# Autodesk Inventor assembly: CL4-300
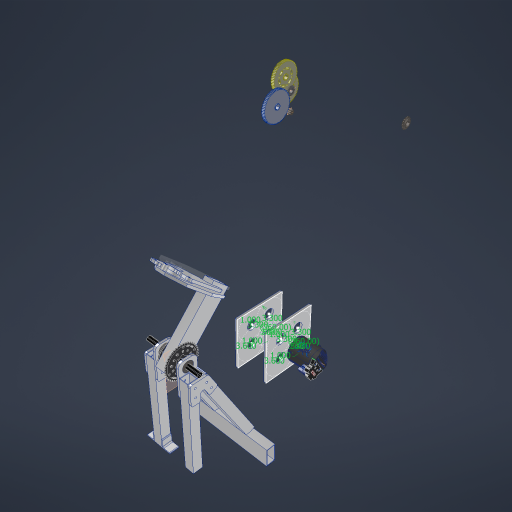
[picture p0: Inventor's stored thumbnail of the model, 512x512]
Saved by Autodesk Inventor 2023.4 (Build 274418000, 418)
## iProperties
Created: 2025-02-04
Part Number: CL4-300
Document SubType Name: Assembly
Designer: brand
Mass: 2767.61 g
Surface Area: 6209.23 cm^2
Volume: 1040.03 cm^3
Density: 2.66107 g/cm^3
Author: brand
## Documents named in this file (15)
- C:\Users\brand\OneDrive\Documents\GitHub\robotics 23\2025-ReefScape---CAD\Climber\CL4\CL4-300.iam
- C:\Users\brand\OneDrive\Documents\GitHub\robotics 23\2025-ReefScape---CAD\Climber\CL4\CL4-200.iam
- C:\Users\brand\OneDrive\Documents\GitHub\robotics 23\2025-ReefScape---CAD\Climber\CL4\CL4-100.iam
- C:\Users\brand\OneDrive\Documents\GitHub\robotics 23\2025-ReefScape---CAD\COMMON PARTS\BEARINGS\0_500_Hex_ID_x_1_125_OD_x_0_313_WD_Flanged_Bearing_v2_217-3875.ipt
- C:\Users\brand\OneDrive\Documents\GitHub\robotics 23\2025-ReefScape---CAD\Climber\CL4\CL4-011.ipt
- C:\Users\brand\OneDrive\Documents\GitHub\robotics 23\2025-ReefScape---CAD\Climber\CL4\CL4-012.ipt
- C:\Users\brand\OneDrive\Documents\GitHub\robotics 23\2025-ReefScape---CAD\Climber\CL4\CL4-013.ipt
- C:\Users\brand\OneDrive\Documents\GitHub\robotics 23\2025-ReefScape---CAD\COMMON PARTS\GEARS\WCP-1006\WCP-1006.ipt
- C:\Users\brand\OneDrive\Documents\GitHub\robotics 23\2025-ReefScape---CAD\COMMON PARTS\GEARS\20dp .5 hex\72t_Aluminum_Spur_Gear_20_DP_1_2_Hex_Bore_217-3576.ipt
- C:\Users\brand\OneDrive\Documents\GitHub\robotics 23\2025-ReefScape---CAD\COMMON PARTS\GEARS\20dp .5 hex\66t_Aluminum_Spur_Gear_20_DP_1_2_Hex_Bore_VersaKeys_217-3223.ipt
- C:\Users\brand\OneDrive\Documents\GitHub\robotics 23\2025-ReefScape---CAD\COMMON PARTS\GEARS\20dp .5 hex\20t_Aluminum_Spur_Gear_20_DP_1_2_Hex_Bore_217-2702.ipt
- C:\Users\brand\OneDrive\Documents\GitHub\robotics 23\2025-ReefScape---CAD\COMMON PARTS\SPROCKETS\25\WCP-0967 42t 25_chain.ipt
- C:\Users\brand\OneDrive\Documents\GitHub\robotics 23\2025-ReefScape---CAD\COMMON PARTS\SPROCKETS\25\14t Steel Double Hub Sprocket (#25 Chain, 12 Hex Bore)\14t Steel Double Hub Sprocket (#25 Chain, 12 Hex Bore).ipt
- C:\Users\brand\OneDrive\Documents\GitHub\robotics 23\2025-ReefScape---CAD\COMMON PARTS\MOTORS\Kracken with Cover and Boards.iam
- C:\Users\brand\OneDrive\Documents\GitHub\robotics 23\2025-ReefScape---CAD\Climber\CL4\CL4-014.ipt
## Components (19 placed, 14 different names)
1. CL4-200:1 [sub-assembly] — Insert:1, Insert:2, Angle:1, Flush:1, Mate:3, Mate:6, Mate:4, Mate:5, Flush:7, Flush:8, Flush:9, Flush:10, Mate:8
2. CL4-100:1 [sub-assembly] — Mate:2, Angle:1, Flush:1, Mate:13, Mate:14
3. 0_500_Hex_ID_x_1_125_OD_x_0_313_WD_Flanged_Bearing_v2_217-3875:1 — Insert:1, Mate:1
4. 0_500_Hex_ID_x_1_125_OD_x_0_313_WD_Flanged_Bearing_v2_217-3875:2 — Insert:2
5. CL4-011:1 — Mate:1, Mate:2
6. CL4-012:1 — Mate:3, Mate:6, Mate:7, Flush:11
7. CL4-013:1 — Mate:4, Flush:7, Flush:8
8. CL4-013:2 — Mate:5, Flush:9, Flush:10
9. CL4-013:3 — Mate:7, Flush:11, Mate:8
10. WCP-1006:1
11. 72t_Aluminum_Spur_Gear_20_DP_1_2_Hex_Bore_217-3576:1
12. 66t_Aluminum_Spur_Gear_20_DP_1_2_Hex_Bore_VersaKeys_217-3223:1
13. 20t_Aluminum_Spur_Gear_20_DP_1_2_Hex_Bore_217-2702:1
14. 66t_Aluminum_Spur_Gear_20_DP_1_2_Hex_Bore_VersaKeys_217-3223:2
15. WCP-0967 42t 25_chain:1 — Mate:13, Mate:14
16. 14t Steel Double Hub Sprocket (#25 Chain, 12 Hex Bore):1
17. Kracken with Cover and Boards:1 [sub-assembly] — Mate:10, Mate:11, Mate:12
18. CL4-014:1
19. CL4-014:2 — Mate:10, Mate:11, Mate:12
## Relationships (24: Mate 14, Flush 7, Insert 2, Angle 1)
- Insert:1: CL4-200:1 ↔ 0_500_Hex_ID_x_1_125_OD_x_0_313_WD_Flanged_Bearing_v2_217-3875:1
- Insert:2: CL4-200:1 ↔ 0_500_Hex_ID_x_1_125_OD_x_0_313_WD_Flanged_Bearing_v2_217-3875:2
- Mate:1: 0_500_Hex_ID_x_1_125_OD_x_0_313_WD_Flanged_Bearing_v2_217-3875:1 ↔ CL4-011:1
- Mate:2: CL4-100:1 ↔ CL4-011:1
- Angle:1 (0 deg): CL4-200:1 ↔ CL4-100:1
- Flush:1: CL4-200:1 ↔ CL4-100:1
- Mate:3: CL4-200:1 ↔ CL4-012:1
- Mate:6: CL4-200:1 ↔ CL4-012:1
- Mate:4: CL4-200:1 ↔ CL4-013:1
- Mate:5: CL4-200:1 ↔ CL4-013:2
- Flush:7: CL4-200:1 ↔ CL4-013:1
- Flush:8: CL4-200:1 ↔ CL4-013:1
- Flush:9: CL4-200:1 ↔ CL4-013:2
- Flush:10: CL4-200:1 ↔ CL4-013:2
- Mate:7: CL4-012:1 ↔ CL4-013:3
- Flush:11: CL4-012:1 ↔ CL4-013:3
- Mate:8: CL4-200:1 ↔ CL4-013:3
- [Flush]: 20t_Aluminum_Spur_Gear_20_DP_1_2_Hex_Bore_217-2702:1 ↔ 66t_Aluminum_Spur_Gear_20_DP_1_2_Hex_Bore_VersaKeys_217-3223:2
- [Mate]: 66t_Aluminum_Spur_Gear_20_DP_1_2_Hex_Bore_VersaKeys_217-3223:1 ↔ 20t_Aluminum_Spur_Gear_20_DP_1_2_Hex_Bore_217-2702:1
- Mate:10: Kracken with Cover and Boards:1 ↔ CL4-014:2
- Mate:11: Kracken with Cover and Boards:1 ↔ CL4-014:2
- Mate:12: Kracken with Cover and Boards:1 ↔ CL4-014:2
- Mate:13: CL4-100:1 ↔ WCP-0967 42t 25_chain:1
- Mate:14: CL4-100:1 ↔ WCP-0967 42t 25_chain:1
